# Autodesk Inventor assembly: elemenet_sprężysty_zaw
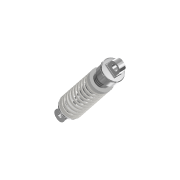
[picture p0: Inventor's stored thumbnail of the model, 180x180]
Saved by Autodesk Inventor 2020.3 (Build 243373000, 373)
## iProperties
Created: 2022-01-11
Part Number: elemenet_sprężysty_zaw
Document SubType Name: Assembly
Designer: patry
Author: patry
## Documents named in this file (5)
- C:\Users\patry\Desktop\Semestr 7\Inzynierka\Projekt inventor\Ariadna_inzynierka\Workspaces\Obszar roboczy\Obszar roboczy\Naped\Amortyzator\elemenet_sprężysty_zaw.iam
- C:\Users\patry\Desktop\Semestr 7\Inzynierka\Projekt inventor\Ariadna_inzynierka\Workspaces\Obszar roboczy\Obszar roboczy\Naped\Amortyzator\Korpus.ipt
- C:\Users\patry\Desktop\Semestr 7\Inzynierka\Projekt inventor\Ariadna_inzynierka\Workspaces\Obszar roboczy\Obszar roboczy\Naped\Amortyzator\Tlok.ipt
- C:\Users\patry\Desktop\Semestr 7\Inzynierka\Projekt inventor\Ariadna_inzynierka\Workspaces\Obszar roboczy\Obszar roboczy\Naped\Amortyzator\Nakretka.ipt
- C:\Users\patry\Desktop\Semestr 7\Inzynierka\Projekt inventor\Ariadna_inzynierka\Workspaces\Obszar roboczy\Obszar roboczy\Naped\Amortyzator\Compress Spring11.ipt
## Components (4 placed, 4 different names)
1. Korpus:1 — Zestawiające:5
2. Tlok:1 — Zestawiające:4, Równoległe:1, Zestawiające:5
3. Nakretka:1
4. Compress Spring1:1 — Zestawiające:4, Równoległe:1
## Relationships (8: Mate 5, Angle 1, CylindricalJoint 1, Flush 1)
- [Mate]: Korpus:1 ↔ Tlok:1
- [Angle] (0 deg): Korpus:1 ↔ Tlok:1
- [Mate]: Korpus:1 ↔ Nakretka:1
- [Mate] (9 mm): Korpus:1 ↔ Nakretka:1
- [CylindricalJoint]: Korpus:1 ↔ Tlok:1
- Zestawiające:4 [Mate]: Tlok:1 ↔ Compress Spring1:1
- Równoległe:1 [Flush]: Tlok:1 ↔ Compress Spring1:1
- Zestawiające:5 [Mate] (52.875 mm): Korpus:1 ↔ Tlok:1
## Named parameters: d83_d6 = -2 mm, d84_d7 = -7.125 mm, d85_d8 = -13 mm, d86_d0 = 0 mm, d87_d1 = 0 deg, d88_d3 = 0 mm, d89_d4 = 9 mm, d90_d5 = 0 deg
